# Autodesk Inventor assembly: Zlozenie
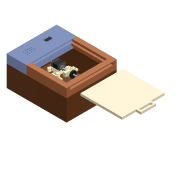
[picture p0: Inventor's stored thumbnail of the model, 180x180]
Saved by Autodesk Inventor 2021 (Build 250183000, 183)
## iProperties
Created: 2022-10-06
Part Number: Zlozenie
Document SubType Name: Assembly
Designer: agnpi
Author: agnpi
## Documents named in this file (22)
- D:\users\agnpi\Desktop\lekcje\SEMESTR VII\INVENTOR 02.11.22\Komponenty_ipt_iam\Zlozenie.iam
- D:\users\agnpi\Desktop\lekcje\SEMESTR VII\INVENTOR 02.11.22\Komponenty_ipt_iam\Podstawa.ipt
- D:\users\agnpi\Desktop\lekcje\SEMESTR VII\INVENTOR 02.11.22\Komponenty_ipt_iam\Duzy_silnik_.ipt
- D:\users\agnpi\Desktop\lekcje\SEMESTR VII\INVENTOR 02.11.22\Komponenty_ipt_iam\Pret_do_duzego_silnika.ipt
- D:\users\agnpi\Desktop\lekcje\SEMESTR VII\INVENTOR 02.11.22\Komponenty_ipt_iam\Uchwyt_wiekszy_silnik_.ipt
- D:\users\agnpi\Desktop\lekcje\SEMESTR VII\INVENTOR 02.11.22\Komponenty_ipt_iam\Zlozenie_prowadnica_na_tlok_nakretka.iam
- D:\users\agnpi\Desktop\lekcje\SEMESTR VII\INVENTOR 02.11.22\Komponenty_ipt_iam\zlozenie_na_strzykawke_.iam
- D:\users\agnpi\Desktop\lekcje\SEMESTR VII\INVENTOR 02.11.22\Komponenty_ipt_iam\maly_silnik_.ipt
- D:\users\agnpi\Desktop\lekcje\SEMESTR VII\INVENTOR 02.11.22\Komponenty_ipt_iam\Zlozenie_na_igle_z_nakretka.iam
- D:\users\agnpi\Desktop\lekcje\SEMESTR VII\INVENTOR 02.11.22\Komponenty_ipt_iam\uchwyt_maly_silnik_.ipt
- D:\users\agnpi\Desktop\lekcje\SEMESTR VII\INVENTOR 02.11.22\Komponenty_ipt_iam\uchwyt_drazki_wersja_2_.ipt
- D:\users\agnpi\Desktop\lekcje\SEMESTR VII\INVENTOR 02.11.22\Komponenty_ipt_iam\plytka_stykowa_mala_.ipt
- D:\users\agnpi\Desktop\lekcje\SEMESTR VII\INVENTOR 02.11.22\Komponenty_ipt_iam\VL6180x_czujnik_.ipt
- D:\users\agnpi\Desktop\lekcje\SEMESTR VII\INVENTOR 02.11.22\Komponenty_ipt_iam\uchwyt_krancowka_alternatywa_2_.ipt
- D:\users\agnpi\Desktop\lekcje\SEMESTR VII\INVENTOR 02.11.22\Komponenty_ipt_iam\krancowka_.ipt
- D:\users\agnpi\Desktop\lekcje\SEMESTR VII\INVENTOR 02.11.22\Komponenty_ipt_iam\gora_altern_krotsza_z_bolcem.ipt
- D:\users\agnpi\Desktop\lekcje\SEMESTR VII\INVENTOR 02.11.22\Komponenty_ipt_iam\pokrywa_krotsza.ipt
- D:\users\agnpi\Desktop\lekcje\SEMESTR VII\INVENTOR 02.11.22\Komponenty_ipt_iam\igla.ipt
- D:\users\agnpi\Desktop\lekcje\SEMESTR VII\INVENTOR 02.11.22\Komponenty_ipt_iam\uchwyt_czujnik.ipt
- D:\users\agnpi\Desktop\lekcje\SEMESTR VII\INVENTOR 02.11.22\Komponenty_ipt_iam\maly_wentylator.ipt
- D:\users\agnpi\Desktop\lekcje\SEMESTR VII\INVENTOR 02.11.22\Komponenty_ipt_iam\plytka_nucleo_zlozenie.iam
- D:\users\agnpi\Desktop\lekcje\SEMESTR VII\INVENTOR 02.11.22\Komponenty_ipt_iam\Kopula+plus_OLED.iam
## Components (28 placed, 21 different names)
1. Podstawa:1 — Mate:1, Mate:2, Mate:3, Mate:7, Mate:8, Mate:9, Mate:10, Mate:11, Mate:12, Mate:16, Mate:17, Mate:18, Mate:22, Mate:23, Mate:27, Mate:28, Mate:32, Mate:34, Mate:36, Mate:37, Mate:42, Mate:43, Flush:13, Mate:44, Mate:47, Mate:55, Mate:56, Mate:57, Mate:58, Flush:60, Mate:62, Mate:63, Mate:64, Mate:65, Mate:66
2. Duzy_silnik_:1 — Rotational:1, Mate:4, Mate:5, Mate:6
3. Pret_do_duzego_silnika:1 — Rotational:1, Cylindrical:1
4. Uchwyt_wiekszy_silnik_:1 — Mate:1, Mate:2, Mate:3, Mate:4, Mate:5, Mate:6
5. Zlozenie_prowadnica_na_tlok_nakretka:1 [sub-assembly] — Cylindrical:1, Angle:4
6. zlozenie_na_strzykawke_:1 [sub-assembly] — Mate:7, Mate:8, Mate:9, Mate:24, Angle:3, Mate:25, Flush:1, Mate:35, Flush:9, Angle:4
7. maly_silnik_:1 — Cylindrical:2, Mate:13, Mate:14, Mate:15
8. Zlozenie_na_igle_z_nakretka:1 [sub-assembly] — Cylindrical:2, Flush:4, Mate:31, Mate:45, Flush:14, Flush:17, Mate:48
9. uchwyt_maly_silnik_:1 — Mate:10, Mate:11, Mate:12, Mate:13, Mate:14, Mate:15, Mate:30
10. uchwyt_drazki_wersja_2_:1 — Mate:16, Mate:17, Mate:18
11. plytka_stykowa_mala_:1 — Mate:22, Mate:23
12. VL6180x_czujnik_:1 — Mate:46, Flush:15, Flush:16, Mate:48
13. VL6180x_czujnik_:2 — Mate:24, Angle:3, Mate:25, Flush:1
14. uchwyt_krancowka_alternatywa_2_:1 — Flush:5, Flush:6, Mate:29, Mate:30, Mate:31, Mate:32
15. uchwyt_krancowka_alternatywa_2_:2 — Flush:2, Mate:26, Flush:3, Flush:4, Mate:27, Mate:28
16. krancowka_:1 — Flush:2, Mate:26, Flush:3
17. krancowka_:2 — Flush:5, Flush:6, Mate:29
18. krancowka_:3 — Flush:7, Mate:33, Flush:8
19. uchwyt_krancowka_alternatywa_2_:3 — Flush:7, Mate:33, Flush:8, Mate:34, Mate:35, Flush:9, Flush:10
20. uchwyt_krancowka_alternatywa_2_:4 — Flush:10, Mate:36, Mate:37, Flush:11, Mate:38, Flush:12
21. krancowka_:4 — Flush:11, Mate:38, Flush:12
22. gora_altern_krotsza_z_bolcem:1 — Mate:42, Mate:43, Flush:13, Mate:44, Slider:1, Mate:55
23. pokrywa_krotsza:1 — Slider:1
24. igla:1 — Mate:45, Flush:14
25. uchwyt_czujnik:1 — Mate:46, Flush:15, Flush:16, Flush:17, Mate:47
26. maly_wentylator:1 — Mate:56, Mate:57, Mate:58
27. plytka_nucleo_zlozenie:1 [sub-assembly] — Flush:60, Mate:62
28. Kopula+plus_OLED:1 [sub-assembly] — Mate:63, Mate:64, Mate:65, Mate:66
## Relationships (75: Mate 51, Flush 18, CylindricalJoint 2, Angle 2, RevoluteJoint 1, TranslationJoint 1)
- Rotational:1 [RevoluteJoint]: Duzy_silnik_:1 ↔ Pret_do_duzego_silnika:1
- Mate:1: Podstawa:1 ↔ Uchwyt_wiekszy_silnik_:1
- Mate:2: Podstawa:1 ↔ Uchwyt_wiekszy_silnik_:1
- Mate:3: Podstawa:1 ↔ Uchwyt_wiekszy_silnik_:1
- Cylindrical:1: Pret_do_duzego_silnika:1 ↔ Zlozenie_prowadnica_na_tlok_nakretka:1
- Mate:4: Duzy_silnik_:1 ↔ Uchwyt_wiekszy_silnik_:1
- Mate:5: Duzy_silnik_:1 ↔ Uchwyt_wiekszy_silnik_:1
- Mate:6: Duzy_silnik_:1 ↔ Uchwyt_wiekszy_silnik_:1
- Mate:7: Podstawa:1 ↔ zlozenie_na_strzykawke_:1
- Mate:8: Podstawa:1 ↔ zlozenie_na_strzykawke_:1
- Mate:9: Podstawa:1 ↔ zlozenie_na_strzykawke_:1
- Cylindrical:2: maly_silnik_:1 ↔ Zlozenie_na_igle_z_nakretka:1
- Mate:10: Podstawa:1 ↔ uchwyt_maly_silnik_:1
- Mate:11: Podstawa:1 ↔ uchwyt_maly_silnik_:1
- Mate:12: Podstawa:1 ↔ uchwyt_maly_silnik_:1
- Mate:13: maly_silnik_:1 ↔ uchwyt_maly_silnik_:1
- Mate:14: maly_silnik_:1 ↔ uchwyt_maly_silnik_:1
- Mate:15: maly_silnik_:1 ↔ uchwyt_maly_silnik_:1
- Mate:16: Podstawa:1 ↔ uchwyt_drazki_wersja_2_:1
- Mate:17: Podstawa:1 ↔ uchwyt_drazki_wersja_2_:1
- Mate:18: Podstawa:1 ↔ uchwyt_drazki_wersja_2_:1
- Mate:22 (5 mm): Podstawa:1 ↔ plytka_stykowa_mala_:1
- Mate:23: Podstawa:1 ↔ plytka_stykowa_mala_:1
- Mate:24: zlozenie_na_strzykawke_:1 ↔ VL6180x_czujnik_:2
- Angle:3 (0 deg): zlozenie_na_strzykawke_:1 ↔ VL6180x_czujnik_:2
- Mate:25 (1 mm): zlozenie_na_strzykawke_:1 ↔ VL6180x_czujnik_:2
- Flush:1: zlozenie_na_strzykawke_:1 ↔ VL6180x_czujnik_:2
- Flush:2: uchwyt_krancowka_alternatywa_2_:2 ↔ krancowka_:1
- Mate:26: uchwyt_krancowka_alternatywa_2_:2 ↔ krancowka_:1
- Flush:3: uchwyt_krancowka_alternatywa_2_:2 ↔ krancowka_:1
- Flush:4: Zlozenie_na_igle_z_nakretka:1 ↔ uchwyt_krancowka_alternatywa_2_:2
- Mate:27: Podstawa:1 ↔ uchwyt_krancowka_alternatywa_2_:2
- Mate:28 (13 mm): Podstawa:1 ↔ uchwyt_krancowka_alternatywa_2_:2
- Flush:5: uchwyt_krancowka_alternatywa_2_:1 ↔ krancowka_:2
- Flush:6: uchwyt_krancowka_alternatywa_2_:1 ↔ krancowka_:2
- Mate:29: uchwyt_krancowka_alternatywa_2_:1 ↔ krancowka_:2
- Mate:30 (8 mm): uchwyt_maly_silnik_:1 ↔ uchwyt_krancowka_alternatywa_2_:1
- Mate:31: Zlozenie_na_igle_z_nakretka:1 ↔ uchwyt_krancowka_alternatywa_2_:1
- Mate:32: Podstawa:1 ↔ uchwyt_krancowka_alternatywa_2_:1
- Flush:7: krancowka_:3 ↔ uchwyt_krancowka_alternatywa_2_:3
- Mate:33: krancowka_:3 ↔ uchwyt_krancowka_alternatywa_2_:3
- Flush:8: krancowka_:3 ↔ uchwyt_krancowka_alternatywa_2_:3
- Mate:34: Podstawa:1 ↔ uchwyt_krancowka_alternatywa_2_:3
- Mate:35: zlozenie_na_strzykawke_:1 ↔ uchwyt_krancowka_alternatywa_2_:3
- Flush:9 (-4 mm): zlozenie_na_strzykawke_:1 ↔ uchwyt_krancowka_alternatywa_2_:3
- Angle:4 (0 deg): Zlozenie_prowadnica_na_tlok_nakretka:1 ↔ zlozenie_na_strzykawke_:1
- Flush:10: uchwyt_krancowka_alternatywa_2_:3 ↔ uchwyt_krancowka_alternatywa_2_:4
- Mate:36: Podstawa:1 ↔ uchwyt_krancowka_alternatywa_2_:4
- Mate:37 (139 mm): Podstawa:1 ↔ uchwyt_krancowka_alternatywa_2_:4
- Flush:11: uchwyt_krancowka_alternatywa_2_:4 ↔ krancowka_:4
- Mate:38: uchwyt_krancowka_alternatywa_2_:4 ↔ krancowka_:4
- Flush:12: uchwyt_krancowka_alternatywa_2_:4 ↔ krancowka_:4
- Mate:42: Podstawa:1 ↔ gora_altern_krotsza_z_bolcem:1
- Mate:43: Podstawa:1 ↔ gora_altern_krotsza_z_bolcem:1
- Flush:13: Podstawa:1 ↔ gora_altern_krotsza_z_bolcem:1
- Mate:44: Podstawa:1 ↔ gora_altern_krotsza_z_bolcem:1
- Slider:1 [TranslationJoint]: gora_altern_krotsza_z_bolcem:1 ↔ pokrywa_krotsza:1
- Mate:45: Zlozenie_na_igle_z_nakretka:1 ↔ igla:1
- Flush:14 (-20 mm): Zlozenie_na_igle_z_nakretka:1 ↔ igla:1
- Mate:46: VL6180x_czujnik_:1 ↔ uchwyt_czujnik:1
- Flush:15: VL6180x_czujnik_:1 ↔ uchwyt_czujnik:1
- Flush:16 (6 mm): VL6180x_czujnik_:1 ↔ uchwyt_czujnik:1
- Flush:17: Zlozenie_na_igle_z_nakretka:1 ↔ uchwyt_czujnik:1
- Mate:47: Podstawa:1 ↔ uchwyt_czujnik:1
- Mate:48 (-5 mm): Zlozenie_na_igle_z_nakretka:1 ↔ VL6180x_czujnik_:1
- Mate:55: Podstawa:1 ↔ gora_altern_krotsza_z_bolcem:1
- Mate:56: Podstawa:1 ↔ maly_wentylator:1
- Mate:57: Podstawa:1 ↔ maly_wentylator:1
- Mate:58: Podstawa:1 ↔ maly_wentylator:1
- Flush:60: Podstawa:1 ↔ plytka_nucleo_zlozenie:1
- Mate:62: Podstawa:1 ↔ plytka_nucleo_zlozenie:1
- Mate:63: Podstawa:1 ↔ Kopula+plus_OLED:1
- Mate:64: Podstawa:1 ↔ Kopula+plus_OLED:1
- Mate:65: Podstawa:1 ↔ Kopula+plus_OLED:1
- Mate:66: Podstawa:1 ↔ Kopula+plus_OLED:1
